# Autodesk Inventor assembly: манипулятор3
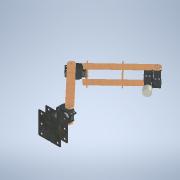
[picture p0: Inventor's stored thumbnail of the model, 180x180]
Saved by Autodesk Inventor 2020.1 (Build 241239000, 239)
## iProperties
Created: 2021-08-18
Part Number: манипулятор3
Document SubType Name: Assembly
Designer: User
Author: User
## Documents named in this file (12)
- C:\Users\Ni3na\Documents\GitHub\avatar-kvantoriada\3D\манипулятор3.iam
- C:\Users\Ni3na\Documents\GitHub\avatar-kvantoriada\3D\основа.ipt
- C:\Users\Ni3na\Documents\GitHub\avatar-kvantoriada\3D\сборка серва 90.iam
- C:\Users\Ni3na\Documents\GitHub\avatar-kvantoriada\3D\сборка серва 45_ЗЕРКАЛО2.iam
- C:\Users\Ni3na\Documents\GitHub\avatar-kvantoriada\3D\Сборка1.iam
- C:\Users\Ni3na\Documents\GitHub\avatar-kvantoriada\3D\уголок.ipt
- C:\Users\Ni3na\Documents\GitHub\avatar-kvantoriada\3D\Сборка2.iam
- C:\Users\Ni3na\Documents\GitHub\avatar-kvantoriada\3D\магнит.ipt
- C:\Users\Ni3na\Documents\GitHub\avatar-kvantoriada\3D\подшипник.iam
- C:\Users\Ni3na\Documents\Inventor\Content Center Files\R2020\ru-RU\AS 1427(08)\AS 1427 - M3 x 8(6) I.ipt
- C:\Users\Ni3na\Documents\Inventor\Content Center Files\R2020\ru-RU\AS 1474(1)\AS 1474 - M3(1).ipt
- C:\Users\Ni3na\Documents\Inventor\Content Center Files\R2020\ru-RU\AS 1427(08)\AS 1427 - M3 x 6(6) I.ipt
## Components (46 placed, 11 different names)
1. основа:1 — Жесткий:1, Жесткий:45, Жесткий:46, Жесткий:47, Жесткий:48
2. основа:2 — Жесткий:1, Жесткий:2, Жесткий:41, Жесткий:42, Жесткий:43, Жесткий:44
3. сборка серва 90:1 [sub-assembly] — Жесткий:2, Жесткий:3
4. сборка серва 45_ЗЕРКАЛО2:1 [sub-assembly] — Жесткий:3, Жесткий:4, Жесткий:31
5. Сборка1:1 [sub-assembly] — Жесткий:4, Жесткий:5, Жесткий:14, Жесткий:15, Жесткий:16, Жесткий:17, Жесткий:22, Жесткий:23, Жесткий:24, Жесткий:25
6. сборка серва 90:2 [sub-assembly] — Жесткий:5, Жесткий:6, Жесткий:32
7. уголок:1 — Жесткий:6, Жесткий:7, Жесткий:33, Жесткий:34, Жесткий:35, Жесткий:36, Жесткий:37, Жесткий:38, Жесткий:39, Жесткий:40
8. Сборка2:1 [sub-assembly] — Жесткий:7, Жесткий:8, Жесткий:18, Жесткий:19, Жесткий:20, Жесткий:21, Жесткий:26, Жесткий:27, Жесткий:28, Жесткий:29
9. сборка серва 90:3 [sub-assembly] — Жесткий:8, Жесткий:9, Жесткий:30
10. сборка серва 90:4 [sub-assembly] — Жесткий:9, Жесткий:10
11. магнит:1 — Жесткий:10
12. AS 1427 Z - метрическая M3 x 8:1 — Жесткий:16
13. AS 1427 Z - метрическая M3 x 8:2 — Жесткий:17
14. AS 1427 Z - метрическая M3 x 8:3 — Жесткий:15
15. AS 1427 Z - метрическая M3 x 8:4 — Жесткий:14
16. AS 1427 Z - метрическая M3 x 8:5 — Жесткий:21
17. AS 1427 Z - метрическая M3 x 8:6 — Жесткий:20
18. AS 1427 Z - метрическая M3 x 8:7 — Жесткий:18
19. AS 1427 Z - метрическая M3 x 8:8 — Жесткий:19
20. AS 1427 Z - метрическая M3 x 8:9 — Жесткий:23
21. AS 1427 Z - метрическая M3 x 8:10 — Жесткий:22
22. AS 1427 Z - метрическая M3 x 8:11 — Жесткий:25
23. AS 1427 Z - метрическая M3 x 8:12 — Жесткий:24
24. AS 1427 Z - метрическая M3 x 8:13 — Жесткий:28
25. AS 1427 Z - метрическая M3 x 8:14 — Жесткий:29
26. AS 1427 Z - метрическая M3 x 8:15 — Жесткий:27
27. AS 1427 Z - метрическая M3 x 8:16 — Жесткий:26
28. подшипник:3 [sub-assembly] — Жесткий:30
29. подшипник:4 [sub-assembly] — Жесткий:31
30. подшипник:5 [sub-assembly] — Жесткий:32
31. AS 1474 - метрическая M3:1 — Жесткий:33
32. AS 1474 - метрическая M3:2 — Жесткий:34
33. AS 1474 - метрическая M3:3 — Жесткий:35
34. AS 1474 - метрическая M3:4 — Жесткий:36
35. AS 1427 Z - метрическая M3 x 6:1 — Жесткий:37
36. AS 1427 Z - метрическая M3 x 6:2 — Жесткий:40
37. AS 1427 Z - метрическая M3 x 6:3 — Жесткий:39
38. AS 1427 Z - метрическая M3 x 6:4 — Жесткий:38
39. AS 1427 Z - метрическая M3 x 8:17 — Жесткий:41
40. AS 1427 Z - метрическая M3 x 8:18 — Жесткий:44
41. AS 1427 Z - метрическая M3 x 8:19 — Жесткий:43
42. AS 1427 Z - метрическая M3 x 8:20 — Жесткий:42
43. AS 1474 - метрическая M3:5 — Жесткий:45
44. AS 1474 - метрическая M3:6 — Жесткий:48
45. AS 1474 - метрическая M3:7 — Жесткий:46
46. AS 1474 - метрическая M3:8 — Жесткий:47
## Relationships (45: WeldJoint 45)
- Жесткий:1 [WeldJoint]: основа:1 ↔ основа:2
- Жесткий:2 [WeldJoint]: основа:2 ↔ сборка серва 90:1
- Жесткий:3 [WeldJoint]: сборка серва 90:1 ↔ сборка серва 45_ЗЕРКАЛО2:1
- Жесткий:4 [WeldJoint]: сборка серва 45_ЗЕРКАЛО2:1 ↔ Сборка1:1
- Жесткий:5 [WeldJoint]: Сборка1:1 ↔ сборка серва 90:2
- Жесткий:6 [WeldJoint]: сборка серва 90:2 ↔ уголок:1
- Жесткий:7 [WeldJoint]: уголок:1 ↔ Сборка2:1
- Жесткий:8 [WeldJoint]: Сборка2:1 ↔ сборка серва 90:3
- Жесткий:9 [WeldJoint]: сборка серва 90:3 ↔ сборка серва 90:4
- Жесткий:10 [WeldJoint]: сборка серва 90:4 ↔ магнит:1
- Жесткий:14 [WeldJoint]: Сборка1:1 ↔ AS 1427 Z - метрическая M3 x 8:4
- Жесткий:15 [WeldJoint]: Сборка1:1 ↔ AS 1427 Z - метрическая M3 x 8:3
- Жесткий:16 [WeldJoint]: Сборка1:1 ↔ AS 1427 Z - метрическая M3 x 8:1
- Жесткий:17 [WeldJoint]: Сборка1:1 ↔ AS 1427 Z - метрическая M3 x 8:2
- Жесткий:18 [WeldJoint]: Сборка2:1 ↔ AS 1427 Z - метрическая M3 x 8:7
- Жесткий:19 [WeldJoint]: Сборка2:1 ↔ AS 1427 Z - метрическая M3 x 8:8
- Жесткий:20 [WeldJoint]: Сборка2:1 ↔ AS 1427 Z - метрическая M3 x 8:6
- Жесткий:21 [WeldJoint]: Сборка2:1 ↔ AS 1427 Z - метрическая M3 x 8:5
- Жесткий:22 [WeldJoint]: Сборка1:1 ↔ AS 1427 Z - метрическая M3 x 8:10
- Жесткий:23 [WeldJoint]: Сборка1:1 ↔ AS 1427 Z - метрическая M3 x 8:9
- Жесткий:24 [WeldJoint]: Сборка1:1 ↔ AS 1427 Z - метрическая M3 x 8:12
- Жесткий:25 [WeldJoint]: Сборка1:1 ↔ AS 1427 Z - метрическая M3 x 8:11
- Жесткий:26 [WeldJoint]: Сборка2:1 ↔ AS 1427 Z - метрическая M3 x 8:16
- Жесткий:27 [WeldJoint]: Сборка2:1 ↔ AS 1427 Z - метрическая M3 x 8:15
- Жесткий:28 [WeldJoint]: Сборка2:1 ↔ AS 1427 Z - метрическая M3 x 8:13
- Жесткий:29 [WeldJoint]: Сборка2:1 ↔ AS 1427 Z - метрическая M3 x 8:14
- Жесткий:30 [WeldJoint]: сборка серва 90:3 ↔ подшипник:3
- Жесткий:31 [WeldJoint]: сборка серва 45_ЗЕРКАЛО2:1 ↔ подшипник:4
- Жесткий:32 [WeldJoint]: сборка серва 90:2 ↔ подшипник:5
- Жесткий:33 [WeldJoint]: уголок:1 ↔ AS 1474 - метрическая M3:1
- Жесткий:34 [WeldJoint]: уголок:1 ↔ AS 1474 - метрическая M3:2
- Жесткий:35 [WeldJoint]: уголок:1 ↔ AS 1474 - метрическая M3:3
- Жесткий:36 [WeldJoint]: уголок:1 ↔ AS 1474 - метрическая M3:4
- Жесткий:37 [WeldJoint]: уголок:1 ↔ AS 1427 Z - метрическая M3 x 6:1
- Жесткий:38 [WeldJoint]: уголок:1 ↔ AS 1427 Z - метрическая M3 x 6:4
- Жесткий:39 [WeldJoint]: уголок:1 ↔ AS 1427 Z - метрическая M3 x 6:3
- Жесткий:40 [WeldJoint]: уголок:1 ↔ AS 1427 Z - метрическая M3 x 6:2
- Жесткий:41 [WeldJoint]: основа:2 ↔ AS 1427 Z - метрическая M3 x 8:17
- Жесткий:42 [WeldJoint]: основа:2 ↔ AS 1427 Z - метрическая M3 x 8:20
- Жесткий:43 [WeldJoint]: основа:2 ↔ AS 1427 Z - метрическая M3 x 8:19
- Жесткий:44 [WeldJoint]: основа:2 ↔ AS 1427 Z - метрическая M3 x 8:18
- Жесткий:45 [WeldJoint]: основа:1 ↔ AS 1474 - метрическая M3:5
- Жесткий:46 [WeldJoint]: основа:1 ↔ AS 1474 - метрическая M3:7
- Жесткий:47 [WeldJoint]: основа:1 ↔ AS 1474 - метрическая M3:8
- Жесткий:48 [WeldJoint]: основа:1 ↔ AS 1474 - метрическая M3:6
